# Autodesk Inventor assembly: Gamepad_Cart
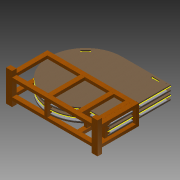
[picture p0: Inventor's stored thumbnail of the model, 180x180]
Saved by Autodesk Inventor 2014 SP1 (Build 180222100, 222)
## iProperties
Created: 2014-02-22
Part Number: Gamepad_Cart
Document SubType Name: Assembly
Designer: tuleu
Author: tuleu
## Documents named in this file (4)
- C:\Users\tuleu\Documents\giant-snes-gamepad\cad\Gamepad_Cart.iam
- C:\Users\tuleu\Documents\giant-snes-gamepad\cad\Gamepad_Left.iam
- C:\Users\tuleu\Documents\giant-snes-gamepad\cad\Gamepad_Right.iam
- C:\Users\tuleu\Documents\giant-snes-gamepad\cad\Cart\Cart.iam
## Components (5 placed, 3 different names)
1. Gamepad_Left:1 [sub-assembly] — Mate:3, Mate:4, Flush:1, Flush:2, Flush:5
2. Gamepad_Left:2 [sub-assembly] — Mate:1, Flush:3, Flush:4, Flush:6
3. Gamepad_Right:1 [sub-assembly] — Mate:3, Flush:1, Flush:6
4. Gamepad_Right:2 [sub-assembly] — Mate:1, Mate:4, Flush:2, Flush:3, Flush:4, Flush:5
5. Cart:1 [sub-assembly]
## Relationships (9: Flush 6, Mate 3)
- Mate:1 (30 mm): Gamepad_Left:2 ↔ Gamepad_Right:2
- Mate:3 (30 mm): Gamepad_Left:1 ↔ Gamepad_Right:1
- Mate:4 (30 mm): Gamepad_Left:1 ↔ Gamepad_Right:2
- Flush:1: Gamepad_Left:1 ↔ Gamepad_Right:1
- Flush:2: Gamepad_Left:1 ↔ Gamepad_Right:2
- Flush:3: Gamepad_Left:2 ↔ Gamepad_Right:2
- Flush:4: Gamepad_Left:2 ↔ Gamepad_Right:2
- Flush:5: Gamepad_Left:1 ↔ Gamepad_Right:2
- Flush:6: Gamepad_Left:2 ↔ Gamepad_Right:1
